# Autodesk Inventor assembly: Minifix&Dowel Joint 111
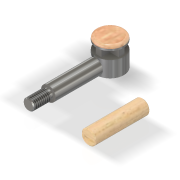
[picture p0: Inventor's stored thumbnail of the model, 180x180]
Saved by Autodesk Inventor 2024 (Build 280153000, 153)
## iProperties
RuleStatus: InUse
AfterAnyParamChange0: Minifix Configuration Control
AfterAnyUserParamChange0: Minifix Configuration Control
Created: 2023-01-09
Part Number: Minifix&Dowel Joint 111
Document SubType Name: Assembly
Designer: sauliusd
Author: sauliusd
## Documents named in this file (6)
- C:\W4INV 2024 Design\PROJECTS\Samples\Macro DEMO\7 Computer Case\Computer Case.iam Smart Hardware\Minifix&Dowel Joint 111\Minifix&Dowel Joint 111.iam
- C:\W4INV 2024 Design\PROJECTS\Samples\Macro DEMO\7 Computer Case\Computer Case.iam Smart Hardware\Minifix&Dowel Joint 111\Minifix&Dowel Joint 11100.ipt
- C:\W4INV 2024 Design\PROJECTS\MODEL STATE LIBRARY COMPONENTS\Minifix D15\Parts\Connecting Pin.ipt
- C:\W4INV 2024 Design\PROJECTS\MODEL STATE LIBRARY COMPONENTS\Minifix D15\Parts\Minifix D15 V4.ipt
- C:\W4INV 2024 Design\PROJECTS\MODEL STATE LIBRARY COMPONENTS\Minifix D15\Parts\Minifix Cap.ipt
- C:\W4INV 2024 Design\PROJECTS\MODEL STATE LIBRARY COMPONENTS\Minifix D15\Parts\Dowel.ipt
## Components (9 placed, 7 different names)
1. Skeleton — Flush:1, Flush:2, Flush:3, Mate:1, Mate:2, Insert:1
2. Dowel — Mate:1, Mate:5
3. Dowel_2 — Mate:2, Mate:6
4. Connecting Pin — Insert:1, Flush:4, Mate:7
5. Minifix CAM — Flush:4, Mate:7, Angle:1, Insert:2
6. Connecting Pin:2
7. Minifix D15 V4:2
8. Minifix Cap — Insert:2
9. Minifix Cap:2
## Component patterns: (1 elements, first: Dowel), (1 elements, first: Dowel_2), (2 elements, first: Connecting Pin + Minifix CAM), CapPattern (2 elements)
## Relationships (12: Mate 5, Flush 4, Insert 2, Angle 1)
- Flush:1: Skeleton
- Flush:2: Skeleton
- Flush:3: Skeleton
- Mate:1: Skeleton ↔ Dowel
- Mate:5: Dowel
- Mate:2: Skeleton ↔ Dowel_2
- Mate:6: Dowel_2
- Insert:1: Skeleton ↔ Connecting Pin
- Flush:4: Connecting Pin ↔ Minifix CAM
- Mate:7: Connecting Pin ↔ Minifix CAM
- Angle:1 (0 deg): Minifix CAM
- Insert:2: Minifix CAM ↔ Minifix Cap
## Named parameters: ContactPatchWidth = 600 mm, ContactPatchHeight = 18 mm, PinLength = 34 mm, ConnectionAngle = 90 deg, Gap = 0 mm, MaxDistBetween = 600 mm, MinDistFromSide1 = 120 mm, MinDistFromSide2 = 60 mm, PlacingSpace = 420 mm, MinDistanceBetween = 90 mm
